# Autodesk Inventor assembly: dovetailAssembly
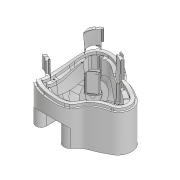
[picture p0: Inventor's stored thumbnail of the model, 180x180]
Saved by Autodesk Inventor 2021 (Build 250183000, 183)
## iProperties
Created: 2020-07-13
Part Number: dovetailAssembly
Document SubType Name: Assembly
Designer: Derm
Author: Derm
## Documents named in this file (3)
- C:\Users\Derm\n95\v7\maskBodyV4Molds\dovetailAssembly.iam
- C:\Users\Derm\n95\v7\maskBodyV4Molds\upperWithDovetails.ipt
- C:\Users\Derm\n95\v7\maskBodyV4Molds\dovetailsV2.ipt
## Components (2 placed, 2 different names)
1. upperWithDovetails:1 — Flush:1, Flush:2
2. dovetailsV2:1 — Flush:1, Flush:2
## Relationships (2: Flush 2)
- Flush:1: upperWithDovetails:1 ↔ dovetailsV2:1
- Flush:2: upperWithDovetails:1 ↔ dovetailsV2:1
